# Autodesk Inventor assembly: PDRUPN50
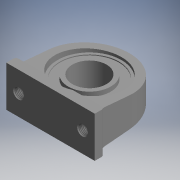
[picture p0: Inventor's stored thumbnail of the model, 180x180]
Saved by Autodesk Inventor 2017.3 (Build 213256000, 256)
## iProperties
Category: PARTsolutions
Company: MISUMI
Part Number: PDRUPN50
Catalog Web Link: www.cadenas.de
Description: PDRUP,PDRUPN-Ball Bearing Units -Pillow Shaped Narrow Type-
Vendor: MISUMI
Document SubType Name: Assembly
Designer: partserver
Manufacturer: MISUMI
Mass: 405.816 g
Surface Area: 647.024 cm^2
Volume: 405.816 cm^3
Density: 1 g/cm^3
Title: PDRUPN50
Author: Cadenas PARTsolutions
Comments: Ball Bearing Units -Pillow Shaped Narrow Type-
PSOL_IDENT_0: {$CADENAS_DATA\23d-libs\misumi\metric\12_bearing_holders\pdrup_asmtab.prj},179 {VTYP=3D},{STYP=ASSTA
PSOL_IDENT_1: B},{NB=PDRUPN50},{LINA=PDRUPN50},{NN=PDRUP,PDRUPN},{DATE=13.11.2019 02:15:11},{GEOMDATE=11.11.2019 0
PSOL_IDENT_2: 8:31:31},{VERSION=},{LINEID=100},{WBVAR=TS},{WBNUMERIC=}  {NB=PDRUPN50},{LINA=PDRUPN50},{KT=DUMMY},{
PSOL_IDENT_3: PN=PDRUPN50},{TYPE=PDRUPN},{MATH=Cast Iron Class No.30},{MATB=52100 Bearing Steel},{MATRS=Nitrile Ru
PSOL_IDENT_4: bber},{MATSS=4137 Alloy Steel},{PRECISION=JIS B 1558/JIS B 1514/JIS B 1559},{OT=-15 ~+100},{TS=2},{T
PSOL_IDENT_5: SALG='1','Lubrication Type' , '2','Oil-Free Type'},{D=50},{JIS=UC210D1},{H=57.2},{L=130},{L1=94},{A=
PSOL_IDENT_6: 60},{M=M16x2},{MD=16},{MPITCH=2.0},{TT=25},{T1=14},{H1=116},{B=51.6},{S=19.0},{CR=35.0},{COR=23.20},
PSOL_IDENT_7: {M1=M8x1},{M1D=8},{M1PITCH=1.00},{M1L=10},{MASS=2600},{RLD=58.8},{RLC=47.0},{LB1=86.48},{LB2=62.4},{
PSOL_IDENT_8: LD1=51},{LD2=33},{LD3=25},{LD4=27.5},{LD5=58.8},{NCL=1.5},{KCL=23.6},{R1=4},{R2=8.0},{PPATH=pdrup/pd
PSOL_IDENT_9: rup_asmtpl.prj}
NB: PDRUPN50
NN: PDRUP,PDRUPN
NT: Ball Bearing Units -Pillow Shaped Narrow Type-
NBSYN: $PN.
LINA: PDRUPN50
CATALOG: Misumi
PN: PDRUPN50
TYPE: PDRUPN
MATH: Cast Iron Class No.30
MATB: 52100 Bearing Steel
MATRS: Nitrile Rubber
MATSS: 4137 Alloy Steel
PRECISION: JIS B 1558/JIS B 1514/JIS B 1559
OT: -15 ~+100
TS: Oil-Free Type
D: 50
JIS: UC210D1
H: 57.2
L: 130
L1: 94
A: 60
M: M16x2
TT: 25
H1: 116
B: 51.6
S: 19
CR: 35
COR: 23.2
M1: M8x1
MASS: 2600
PPATH: pdrup/pdrup_asmtpl.prj
SUPPLIER: MISUMI
ARTICLENO: PDRUPN50
BOMINFO: PDRUPN50
CREATOR: CADENAS GmbH
## Documents named in this file (3)
- e:\temp\worker_19\temp\exporttempdir_7668_338_XgOz2\format_0\PDRUPN50.iam
- e:\temp\worker_19\temp\exporttempdir_7668_338_XgOz2\format_0\PDRUPN50_b.ipt
- e:\temp\worker_19\temp\exporttempdir_7668_338_XgOz2\format_0\SET-SCREW8-10.ipt
## Components (3 placed, 2 different names)
1. PDRUPN50_b:1 — cp1_XY@1 <-> CP_XY@2, cp1_Z@1 <-> CP_Z@2, cp1_YZ@1 <-> CP_YZ@2, cp2_XY@1 <-> CP_XY@3, cp2_Z@1 <-> CP_Z@3, cp2_YZ@1 <-> CP_YZ@3
2. SET-SCREW8-10:1 — cp1_XY@1 <-> CP_XY@2, cp1_Z@1 <-> CP_Z@2, cp1_YZ@1 <-> CP_YZ@2
3. SET-SCREW8-10:2 — cp2_XY@1 <-> CP_XY@3, cp2_Z@1 <-> CP_Z@3, cp2_YZ@1 <-> CP_YZ@3
## Relationships (6: Mate 4, Angle 2)
- cp1_XY@1 <-> CP_XY@2 [Mate]: PDRUPN50_b:1 ↔ SET-SCREW8-10:1
- cp1_Z@1 <-> CP_Z@2 [Mate]: PDRUPN50_b:1 ↔ SET-SCREW8-10:1
- cp1_YZ@1 <-> CP_YZ@2 [Angle] (0 deg): PDRUPN50_b:1 ↔ SET-SCREW8-10:1
- cp2_XY@1 <-> CP_XY@3 [Mate]: PDRUPN50_b:1 ↔ SET-SCREW8-10:2
- cp2_Z@1 <-> CP_Z@3 [Mate]: PDRUPN50_b:1 ↔ SET-SCREW8-10:2
- cp2_YZ@1 <-> CP_YZ@3 [Angle] (0 deg): PDRUPN50_b:1 ↔ SET-SCREW8-10:2
